# Autodesk Inventor assembly: Rover_2.0
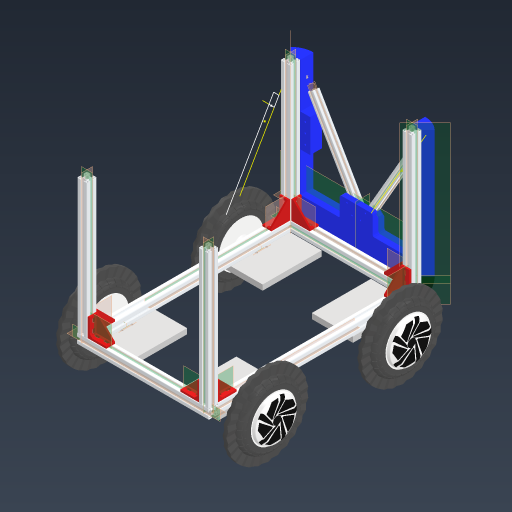
[picture p0: Inventor's stored thumbnail of the model, 512x512]
Saved by Autodesk Inventor 2023.2 (Build 272271030, 271C)
## iProperties
Created: 2025-08-19
Part Number: Rover_2.0
Document SubType Name: Assembly
Designer: Олег Коноваленко
Author: Олег Коноваленко
## Documents named in this file (6)
- D:\!Rover\Rover\Rover_construction\Rover_2.0.iam
- D:\!Rover\Rover\Rover_construction\Профиль 30x30\Грубый профиль_30x30.ipt
- D:\!Rover\Rover\Rover_construction\Задняя стенка.iam
- C:\Users\I9232\Downloads\SNSS.30.70.06.-Uglovoy-alyuminievyy-soedinitel-30kh60_-paz-8_X04_\SNSS.30.70.06.-Uglovoy-alyuminievyy-soedinitel-30kh60_-paz-8_X04_.ipt
- D:\!Rover\Rover\Rover_construction\Крепление мотора.iam
- D:\!Rover\Rover\Rover_construction\Motor, BLDC, Hoverboard Wheel, 8.0in.ipt
## Components (25 placed, 5 different names)
1. SNSS.30.70.06.-Uglovoy-alyuminievyy-soedinitel-30kh60_-paz-8_X04_:1 — Совмещение:51, Совмещение:52, Совмещение:70
2. SNSS.30.70.06.-Uglovoy-alyuminievyy-soedinitel-30kh60_-paz-8_X04_:2 — Совмещение:64, Совмещение:65, Заподлицо:32
3. SNSS.30.70.06.-Uglovoy-alyuminievyy-soedinitel-30kh60_-paz-8_X04_:3 — Совмещение:56, Совмещение:57, Совмещение:68
4. SNSS.30.70.06.-Uglovoy-alyuminievyy-soedinitel-30kh60_-paz-8_X04_:4 — Совмещение:58, Совмещение:59, Совмещение:69
5. SNSS.30.70.06.-Uglovoy-alyuminievyy-soedinitel-30kh60_-paz-8_X04_:5 — Совмещение:61, Совмещение:62, Совмещение:71
6. SNSS.30.70.06.-Uglovoy-alyuminievyy-soedinitel-30kh60_-paz-8_X04_:6 — Совмещение:50, Совмещение:67, Заподлицо:31
7. SNSS.30.70.06.-Uglovoy-alyuminievyy-soedinitel-30kh60_-paz-8_X04_:7 — Совмещение:55, Совмещение:63, Заподлицо:33
8. SNSS.30.70.06.-Uglovoy-alyuminievyy-soedinitel-30kh60_-paz-8_X04_:8 — Совмещение:60, Совмещение:66, Заподлицо:30
9. Крепление мотора:1 [sub-assembly] — Совмещение:73, Заподлицо:37, Заподлицо:38, Совмещение:82, Совмещение:83, Совмещение:84
10. Крепление мотора:2 [sub-assembly] — Совмещение:75, Заподлицо:34, Заподлицо:40, Совмещение:76, Совмещение:77, Совмещение:78
11. Крепление мотора:3 [sub-assembly] — Совмещение:72, Заподлицо:36, Заподлицо:39, Совмещение:79, Совмещение:80, Совмещение:81
12. Крепление мотора:4 [sub-assembly] — Совмещение:74, Заподлицо:35, Заподлицо:41, Совмещение:85, Совмещение:86, Совмещение:87
13. Motor, BLDC, Hoverboard Wheel, 8.0in:1 — Совмещение:76, Совмещение:77, Совмещение:78
14. Motor, BLDC, Hoverboard Wheel, 8.0in:2 — Совмещение:79, Совмещение:80, Совмещение:81
15. Motor, BLDC, Hoverboard Wheel, 8.0in:3 — Совмещение:85, Совмещение:86, Совмещение:87
16. Motor, BLDC, Hoverboard Wheel, 8.0in:4 — Совмещение:82, Совмещение:83, Совмещение:84
17. Задняя стенка:1 [sub-assembly] — Совмещение:88, Заподлицо:42, Заподлицо:43
18. Грубый профиль_30x30:1 — Заподлицо:15, Совмещение:40, Совмещение:41, Заподлицо:17, Заподлицо:18, Заподлицо:21, Совмещение:57, Совмещение:62, Совмещение:68, Совмещение:71, Совмещение:74, Совмещение:75, Заподлицо:34, Заподлицо:35
19. Грубый профиль_30x30:2 — Совмещение:45, Заподлицо:26, Заподлицо:27, Совмещение:56, Совмещение:66
20. Грубый профиль_30x30:3 — Совмещение:46, Заподлицо:28, Заподлицо:29, Совмещение:50, Совмещение:58, Заподлицо:42, Заподлицо:43
21. Грубый профиль_30x30:4 — Совмещение:40, Заподлицо:18, Заподлицо:20, Заподлицо:21, Совмещение:45, Совмещение:46, Заподлицо:26, Заподлицо:27, Заподлицо:28, Заподлицо:29, Совмещение:60, Совмещение:67, Заподлицо:30, Заподлицо:31, Заподлицо:39, Заподлицо:40, Совмещение:88
22. Грубый профиль_30x30:5 — Совмещение:42, Заподлицо:16, Заподлицо:19, Заподлицо:20, Совмещение:52, Совмещение:59, Совмещение:69, Совмещение:70, Совмещение:72, Совмещение:73, Заподлицо:36, Заподлицо:37
23. Грубый профиль_30x30:6 — Совмещение:44, Заподлицо:22, Заподлицо:23, Совмещение:51, Совмещение:64
24. Грубый профиль_30x30:7 — Совмещение:43, Заподлицо:24, Заподлицо:25, Совмещение:55, Совмещение:61
25. Грубый профиль_30x30:8 — Совмещение:41, Совмещение:42, Заподлицо:16, Заподлицо:17, Заподлицо:19, Совмещение:43, Совмещение:44, Заподлицо:22, Заподлицо:23, Заподлицо:24, Заподлицо:25, Совмещение:63, Совмещение:65, Заподлицо:32, Заподлицо:33, Заподлицо:38, Заподлицо:41
## Relationships (77: Mate 48, Flush 29)
- Совмещение:16 [Mate]
- Совмещение:17 [Mate]
- Заподлицо:15 [Flush]: Грубый профиль_30x30:1
- Совмещение:38 [Mate]
- Совмещение:39 [Mate]
- Совмещение:40 [Mate]: Грубый профиль_30x30:1 ↔ Грубый профиль_30x30:4
- Совмещение:41 [Mate]: Грубый профиль_30x30:1 ↔ Грубый профиль_30x30:8
- Совмещение:42 [Mate]: Грубый профиль_30x30:5 ↔ Грубый профиль_30x30:8
- Заподлицо:16 [Flush]: Грубый профиль_30x30:5 ↔ Грубый профиль_30x30:8
- Заподлицо:17 [Flush]: Грубый профиль_30x30:1 ↔ Грубый профиль_30x30:8
- Заподлицо:18 [Flush]: Грубый профиль_30x30:1 ↔ Грубый профиль_30x30:4
- Заподлицо:19 [Flush]: Грубый профиль_30x30:5 ↔ Грубый профиль_30x30:8
- Заподлицо:20 [Flush]: Грубый профиль_30x30:4 ↔ Грубый профиль_30x30:5
- Заподлицо:21 [Flush]: Грубый профиль_30x30:1 ↔ Грубый профиль_30x30:4
- Совмещение:43 [Mate]: Грубый профиль_30x30:7 ↔ Грубый профиль_30x30:8
- Совмещение:44 [Mate]: Грубый профиль_30x30:6 ↔ Грубый профиль_30x30:8
- Совмещение:45 [Mate]: Грубый профиль_30x30:2 ↔ Грубый профиль_30x30:4
- Совмещение:46 [Mate]: Грубый профиль_30x30:3 ↔ Грубый профиль_30x30:4
- Заподлицо:22 [Flush]: Грубый профиль_30x30:6 ↔ Грубый профиль_30x30:8
- Заподлицо:23 [Flush]: Грубый профиль_30x30:6 ↔ Грубый профиль_30x30:8
- Заподлицо:24 [Flush]: Грубый профиль_30x30:7 ↔ Грубый профиль_30x30:8
- Заподлицо:25 [Flush]: Грубый профиль_30x30:7 ↔ Грубый профиль_30x30:8
- Заподлицо:26 [Flush]: Грубый профиль_30x30:2 ↔ Грубый профиль_30x30:4
- Заподлицо:27 [Flush]: Грубый профиль_30x30:2 ↔ Грубый профиль_30x30:4
- Заподлицо:28 [Flush]: Грубый профиль_30x30:3 ↔ Грубый профиль_30x30:4
- Заподлицо:29 [Flush]: Грубый профиль_30x30:3 ↔ Грубый профиль_30x30:4
- Совмещение:50 [Mate]: SNSS.30.70.06.-Uglovoy-alyuminievyy-soedinitel-30kh60_-paz-8_X04_:6 ↔ Грубый профиль_30x30:3
- Совмещение:51 [Mate]: SNSS.30.70.06.-Uglovoy-alyuminievyy-soedinitel-30kh60_-paz-8_X04_:1 ↔ Грубый профиль_30x30:6
- Совмещение:52 [Mate]: SNSS.30.70.06.-Uglovoy-alyuminievyy-soedinitel-30kh60_-paz-8_X04_:1 ↔ Грубый профиль_30x30:5
- Совмещение:55 [Mate]: SNSS.30.70.06.-Uglovoy-alyuminievyy-soedinitel-30kh60_-paz-8_X04_:7 ↔ Грубый профиль_30x30:7
- Совмещение:56 [Mate]: SNSS.30.70.06.-Uglovoy-alyuminievyy-soedinitel-30kh60_-paz-8_X04_:3 ↔ Грубый профиль_30x30:2
- Совмещение:57 [Mate]: SNSS.30.70.06.-Uglovoy-alyuminievyy-soedinitel-30kh60_-paz-8_X04_:3 ↔ Грубый профиль_30x30:1
- Совмещение:58 [Mate]: SNSS.30.70.06.-Uglovoy-alyuminievyy-soedinitel-30kh60_-paz-8_X04_:4 ↔ Грубый профиль_30x30:3
- Совмещение:59 [Mate]: SNSS.30.70.06.-Uglovoy-alyuminievyy-soedinitel-30kh60_-paz-8_X04_:4 ↔ Грубый профиль_30x30:5
- Совмещение:60 [Mate]: SNSS.30.70.06.-Uglovoy-alyuminievyy-soedinitel-30kh60_-paz-8_X04_:8 ↔ Грубый профиль_30x30:4
- Совмещение:61 [Mate]: SNSS.30.70.06.-Uglovoy-alyuminievyy-soedinitel-30kh60_-paz-8_X04_:5 ↔ Грубый профиль_30x30:7
- Совмещение:62 [Mate]: SNSS.30.70.06.-Uglovoy-alyuminievyy-soedinitel-30kh60_-paz-8_X04_:5 ↔ Грубый профиль_30x30:1
- Совмещение:63 [Mate]: SNSS.30.70.06.-Uglovoy-alyuminievyy-soedinitel-30kh60_-paz-8_X04_:7 ↔ Грубый профиль_30x30:8
- Совмещение:64 [Mate]: SNSS.30.70.06.-Uglovoy-alyuminievyy-soedinitel-30kh60_-paz-8_X04_:2 ↔ Грубый профиль_30x30:6
- Совмещение:65 [Mate]: SNSS.30.70.06.-Uglovoy-alyuminievyy-soedinitel-30kh60_-paz-8_X04_:2 ↔ Грубый профиль_30x30:8
- Совмещение:66 [Mate]: SNSS.30.70.06.-Uglovoy-alyuminievyy-soedinitel-30kh60_-paz-8_X04_:8 ↔ Грубый профиль_30x30:2
- Совмещение:67 [Mate]: SNSS.30.70.06.-Uglovoy-alyuminievyy-soedinitel-30kh60_-paz-8_X04_:6 ↔ Грубый профиль_30x30:4
- Совмещение:68 [Mate]: SNSS.30.70.06.-Uglovoy-alyuminievyy-soedinitel-30kh60_-paz-8_X04_:3 ↔ Грубый профиль_30x30:1
- Заподлицо:30 [Flush]: SNSS.30.70.06.-Uglovoy-alyuminievyy-soedinitel-30kh60_-paz-8_X04_:8 ↔ Грубый профиль_30x30:4
- Заподлицо:31 [Flush]: SNSS.30.70.06.-Uglovoy-alyuminievyy-soedinitel-30kh60_-paz-8_X04_:6 ↔ Грубый профиль_30x30:4
- Совмещение:69 [Mate]: SNSS.30.70.06.-Uglovoy-alyuminievyy-soedinitel-30kh60_-paz-8_X04_:4 ↔ Грубый профиль_30x30:5
- Совмещение:70 [Mate]: SNSS.30.70.06.-Uglovoy-alyuminievyy-soedinitel-30kh60_-paz-8_X04_:1 ↔ Грубый профиль_30x30:5
- Заподлицо:32 [Flush]: SNSS.30.70.06.-Uglovoy-alyuminievyy-soedinitel-30kh60_-paz-8_X04_:2 ↔ Грубый профиль_30x30:8
- Заподлицо:33 [Flush]: SNSS.30.70.06.-Uglovoy-alyuminievyy-soedinitel-30kh60_-paz-8_X04_:7 ↔ Грубый профиль_30x30:8
- Совмещение:71 [Mate]: SNSS.30.70.06.-Uglovoy-alyuminievyy-soedinitel-30kh60_-paz-8_X04_:5 ↔ Грубый профиль_30x30:1
- Совмещение:72 [Mate]: Крепление мотора:3 ↔ Грубый профиль_30x30:5
- Совмещение:73 [Mate]: Крепление мотора:1 ↔ Грубый профиль_30x30:5
- Совмещение:74 [Mate]: Крепление мотора:4 ↔ Грубый профиль_30x30:1
- Совмещение:75 [Mate]: Крепление мотора:2 ↔ Грубый профиль_30x30:1
- Заподлицо:34 [Flush]: Крепление мотора:2 ↔ Грубый профиль_30x30:1
- Заподлицо:35 [Flush]: Крепление мотора:4 ↔ Грубый профиль_30x30:1
- Заподлицо:36 [Flush]: Крепление мотора:3 ↔ Грубый профиль_30x30:5
- Заподлицо:37 [Flush]: Крепление мотора:1 ↔ Грубый профиль_30x30:5
- Заподлицо:38 [Flush] (30 mm): Крепление мотора:1 ↔ Грубый профиль_30x30:8
- Заподлицо:39 [Flush] (30 mm): Крепление мотора:3 ↔ Грубый профиль_30x30:4
- Заподлицо:40 [Flush] (30 mm): Крепление мотора:2 ↔ Грубый профиль_30x30:4
- Заподлицо:41 [Flush] (30 mm): Крепление мотора:4 ↔ Грубый профиль_30x30:8
- Совмещение:76 [Mate]: Крепление мотора:2 ↔ Motor, BLDC, Hoverboard Wheel, 8.0in:1
- Совмещение:77 [Mate]: Крепление мотора:2 ↔ Motor, BLDC, Hoverboard Wheel, 8.0in:1
- Совмещение:78 [Mate]: Крепление мотора:2 ↔ Motor, BLDC, Hoverboard Wheel, 8.0in:1
- Совмещение:79 [Mate]: Крепление мотора:3 ↔ Motor, BLDC, Hoverboard Wheel, 8.0in:2
- Совмещение:80 [Mate]: Крепление мотора:3 ↔ Motor, BLDC, Hoverboard Wheel, 8.0in:2
- Совмещение:81 [Mate]: Крепление мотора:3 ↔ Motor, BLDC, Hoverboard Wheel, 8.0in:2
- Совмещение:82 [Mate]: Крепление мотора:1 ↔ Motor, BLDC, Hoverboard Wheel, 8.0in:4
- Совмещение:83 [Mate]: Крепление мотора:1 ↔ Motor, BLDC, Hoverboard Wheel, 8.0in:4
- Совмещение:84 [Mate]: Крепление мотора:1 ↔ Motor, BLDC, Hoverboard Wheel, 8.0in:4
- Совмещение:85 [Mate]: Крепление мотора:4 ↔ Motor, BLDC, Hoverboard Wheel, 8.0in:3
- Совмещение:86 [Mate]: Крепление мотора:4 ↔ Motor, BLDC, Hoverboard Wheel, 8.0in:3
- Совмещение:87 [Mate]: Крепление мотора:4 ↔ Motor, BLDC, Hoverboard Wheel, 8.0in:3
- Совмещение:88 [Mate]: Задняя стенка:1 ↔ Грубый профиль_30x30:4
- Заподлицо:42 [Flush]: Задняя стенка:1 ↔ Грубый профиль_30x30:3
- Заподлицо:43 [Flush]: Задняя стенка:1 ↔ Грубый профиль_30x30:3
